# Autodesk Inventor assembly: proteox_fridge
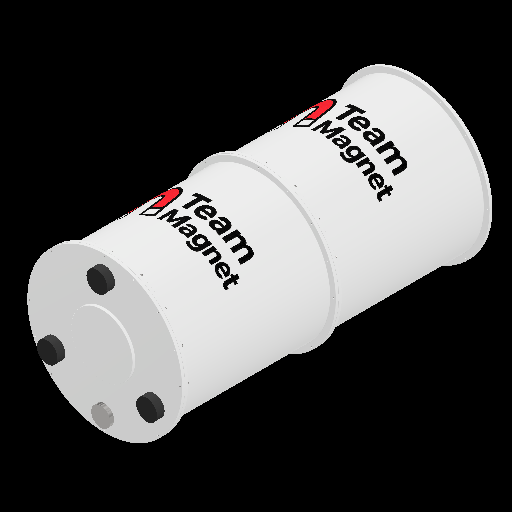
[picture p0: Inventor's stored thumbnail of the model, 512x512]
Saved by Autodesk Inventor 2026.1 (Build 301233000, 233)
## iProperties
Created: 2025-09-17
Part Number: proteox_fridge
Document SubType Name: Assembly
Designer: drago
Author: drago
## Documents named in this file (6)
- C:\Users\drago\Desktop\_QIST4500_Multidisciplinary_Team_Project\Proteox MX magnet positioner CAD\proteox_mx_fridge\proteox_fridge.iam
- C:\Users\drago\Desktop\_QIST4500_Multidisciplinary_Team_Project\Proteox MX magnet positioner CAD\proteox_mx_fridge\proteox_tube.ipt
- C:\Users\drago\Desktop\_QIST4500_Multidisciplinary_Team_Project\Proteox MX magnet positioner CAD\proteox_mx_fridge\proteox_bottom_lid.ipt
- C:\Users\drago\Documents\Inventor\Content Center Files\R2026\en-US\AS 1420\AS 1420 - 1973 - M5 x 25.ipt
- C:\Users\drago\Documents\Inventor\Content Center Files\R2026\en-US\AS 1237 (4.1)\AS 1237 - 5 mm(2).ipt
- C:\Users\drago\Documents\Inventor\Content Center Files\R2026\en-US\CNS 4473\CNS 4473 - M 5 x 0.8.ipt
## Components (47 placed, 5 different names)
1. proteox_tube:1 — Mate:1, Mate:2, Mate:5, Mate:7, Mate:8, Mate:10, Mate:15, Mate:16, Mate:19, Mate:22, Mate:23, Mate:24, Mate:27, Mate:30, Mate:32
2. proteox_tube:2 — Mate:3, Angle:2, Mate:5, Mate:6, Mate:11, Mate:12, Mate:14, Mate:17, Mate:18, Mate:20, Mate:21, Mate:25, Mate:26, Mate:28, Mate:29, Mate:31
3. proteox_bottom_lid:1 — Mate:4, Angle:1, Mate:6
4. AS 1237 (4.1) 5 mm:17 — Mate:19, Angle:7, Mate:22, Mate:37
5. AS 1237 (4.1) 5 mm:18 — Mate:15, Angle:8, Mate:24, Mate:33
6. AS 1237 (4.1) 5 mm:19 — Mate:17, Angle:9, Mate:26, Mate:34
7. AS 1237 (4.1) 5 mm:20 — Mate:18, Mate:25, Angle:11, Mate:36
8. AS 1237 (4.1) 5 mm:21 — Mate:16, Mate:23, Angle:12, Mate:35
9. AS 1237 (4.1) 5 mm:22 — Mate:20, Mate:21, Angle:10, Mate:38
10. CNS 4473 M 5:1 — Mate:27, Mate:37, Angle:13
11. CNS 4473 M 5:2 — Mate:28, Mate:38, Angle:14
12. CNS 4473 M 5:3 — Mate:29, Mate:34, Angle:15
13. CNS 4473 M 5:4 — Mate:31, Mate:36, Angle:16
14. CNS 4473 M 5:5 — Mate:30, Mate:33, Angle:17
15. CNS 4473 M 5:6 — Mate:32, Mate:35, Angle:18
16. AS 1420 - Metric M5 x 25:1 — Mate:8, Mate:9, Angle:3
17. AS 1237 (4.1) 5 mm:1 — Mate:7, Mate:9, Mate:10, Angle:4
18. AS 1420 - Metric M5 x 25:2
19. AS 1237 (4.1) 5 mm:2
20. AS 1420 - Metric M5 x 25:3
21. AS 1237 (4.1) 5 mm:3
22. AS 1420 - Metric M5 x 25:4
23. AS 1237 (4.1) 5 mm:4
24. AS 1420 - Metric M5 x 25:5
25. AS 1237 (4.1) 5 mm:5
26. AS 1420 - Metric M5 x 25:6
27. AS 1237 (4.1) 5 mm:6
28. AS 1420 - Metric M5 x 25:7
29. AS 1237 (4.1) 5 mm:7
30. AS 1420 - Metric M5 x 25:8
31. AS 1237 (4.1) 5 mm:8
32. AS 1237 (4.1) 5 mm:9 — Mate:11, Angle:6, Mate:13, Mate:14
33. AS 1420 - Metric M5 x 25:9 — Mate:12, Angle:5, Mate:13
34. AS 1237 (4.1) 5 mm:10
35. AS 1420 - Metric M5 x 25:10
36. AS 1237 (4.1) 5 mm:11
37. AS 1420 - Metric M5 x 25:11
38. AS 1237 (4.1) 5 mm:12
39. AS 1420 - Metric M5 x 25:12
40. AS 1237 (4.1) 5 mm:13
41. AS 1420 - Metric M5 x 25:13
42. AS 1237 (4.1) 5 mm:14
43. AS 1420 - Metric M5 x 25:14
44. AS 1237 (4.1) 5 mm:15
45. AS 1420 - Metric M5 x 25:15
46. AS 1237 (4.1) 5 mm:16
47. AS 1420 - Metric M5 x 25:16
## Component patterns: (8 elements, first: AS 1420 - Metric M5 x 25:1 + AS 1237 (4.1) 5 mm:1), (8 elements, first: AS 1237 (4.1) 5 mm:9 + AS 1420 - Metric M5 x 25:9)
## Relationships (56: Mate 38, Angle 18)
- Mate:1: proteox_tube:1
- Mate:2: proteox_tube:1
- Mate:3: proteox_tube:2
- Mate:4: proteox_bottom_lid:1
- Angle:1 (0 deg): proteox_bottom_lid:1
- Angle:2 (0 deg): proteox_tube:2
- Mate:5: proteox_tube:1 ↔ proteox_tube:2
- Mate:6: proteox_tube:2 ↔ proteox_bottom_lid:1
- Mate:7: proteox_tube:1 ↔ AS 1237 (4.1) 5 mm:1
- Mate:8: proteox_tube:1 ↔ AS 1420 - Metric M5 x 25:1
- Mate:9: AS 1420 - Metric M5 x 25:1 ↔ AS 1237 (4.1) 5 mm:1
- Mate:10: proteox_tube:1 ↔ AS 1237 (4.1) 5 mm:1
- Angle:3 (0 deg): AS 1420 - Metric M5 x 25:1
- Angle:4 (0 deg): AS 1237 (4.1) 5 mm:1
- Mate:11: proteox_tube:2 ↔ AS 1237 (4.1) 5 mm:9
- Mate:12: proteox_tube:2 ↔ AS 1420 - Metric M5 x 25:9
- Angle:5 (0 deg): AS 1420 - Metric M5 x 25:9
- Angle:6 (0 deg): AS 1237 (4.1) 5 mm:9
- Mate:13: AS 1237 (4.1) 5 mm:9 ↔ AS 1420 - Metric M5 x 25:9
- Mate:14: proteox_tube:2 ↔ AS 1237 (4.1) 5 mm:9
- Mate:15: proteox_tube:1 ↔ AS 1237 (4.1) 5 mm:18
- Mate:16: proteox_tube:1 ↔ AS 1237 (4.1) 5 mm:21
- Mate:17: proteox_tube:2 ↔ AS 1237 (4.1) 5 mm:19
- Mate:18: proteox_tube:2 ↔ AS 1237 (4.1) 5 mm:20
- Mate:19: proteox_tube:1 ↔ AS 1237 (4.1) 5 mm:17
- Mate:20: proteox_tube:2 ↔ AS 1237 (4.1) 5 mm:22
- Angle:7 (0 deg): AS 1237 (4.1) 5 mm:17
- Angle:8 (0 deg): AS 1237 (4.1) 5 mm:18
- Angle:9 (0 deg): AS 1237 (4.1) 5 mm:19
- Mate:21: proteox_tube:2 ↔ AS 1237 (4.1) 5 mm:22
- Mate:22: proteox_tube:1 ↔ AS 1237 (4.1) 5 mm:17
- Angle:10 (0 deg): AS 1237 (4.1) 5 mm:22
- Mate:23: proteox_tube:1 ↔ AS 1237 (4.1) 5 mm:21
- Mate:24: proteox_tube:1 ↔ AS 1237 (4.1) 5 mm:18
- Mate:25: proteox_tube:2 ↔ AS 1237 (4.1) 5 mm:20
- Mate:26: proteox_tube:2 ↔ AS 1237 (4.1) 5 mm:19
- Angle:11 (0 deg): AS 1237 (4.1) 5 mm:20
- Angle:12 (0 deg): AS 1237 (4.1) 5 mm:21
- Mate:27: proteox_tube:1 ↔ CNS 4473 M 5:1
- Mate:28: proteox_tube:2 ↔ CNS 4473 M 5:2
- Mate:29: proteox_tube:2 ↔ CNS 4473 M 5:3
- Mate:30: proteox_tube:1 ↔ CNS 4473 M 5:5
- Mate:31: proteox_tube:2 ↔ CNS 4473 M 5:4
- Mate:32: proteox_tube:1 ↔ CNS 4473 M 5:6
- Mate:33: AS 1237 (4.1) 5 mm:18 ↔ CNS 4473 M 5:5
- Mate:34: AS 1237 (4.1) 5 mm:19 ↔ CNS 4473 M 5:3
- Mate:35: AS 1237 (4.1) 5 mm:21 ↔ CNS 4473 M 5:6
- Mate:36: AS 1237 (4.1) 5 mm:20 ↔ CNS 4473 M 5:4
- Mate:37: AS 1237 (4.1) 5 mm:17 ↔ CNS 4473 M 5:1
- Mate:38: AS 1237 (4.1) 5 mm:22 ↔ CNS 4473 M 5:2
- Angle:13 (0 deg): CNS 4473 M 5:1
- Angle:14 (0 deg): CNS 4473 M 5:2
- Angle:15 (0 deg): CNS 4473 M 5:3
- Angle:16 (0 deg): CNS 4473 M 5:4
- Angle:17 (0 deg): CNS 4473 M 5:5
- Angle:18 (0 deg): CNS 4473 M 5:6
